# Autodesk Inventor assembly: DayLightGlow_DisplayPanel
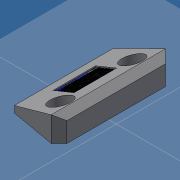
[picture p0: Inventor's stored thumbnail of the model, 180x180]
Saved by Autodesk Inventor 2019 (Build 230136000, 136)
## iProperties
Created: 2019-01-06
Part Number: DayLightGlow_DisplayPanel
Material: Generisch
Document SubType Name: Assembly
Designer: Stefan
Mass: 14.7018 g
Surface Area: 181.288 cm^2
Volume: 14.7018 cm^3
Density: 1 g/cm^3
Author: Stefan
## Documents named in this file (3)
- C:\Users\User\Documents\Inventor\DayLightGlow\DayLightGlow_DisplayPanel.iam
- C:\Users\User\Documents\Inventor\DayLightGlow\DayLightGlow_DisplayPanel.ipt
- C:\Users\User\Documents\Inventor\DayLightGlow\Geekcreit 1.3 Inch 4Pin.ipt
## Components (2 placed, 2 different names)
1. DayLightGlow_DisplayPanel:1 — Passend:1, Passend:2, Passend:3
2. Geekcreit 1.3 Inch 4Pin:1 — Passend:1, Passend:2, Passend:3
## Relationships (3: Mate 3)
- Passend:1 [Mate]: DayLightGlow_DisplayPanel:1 ↔ Geekcreit 1.3 Inch 4Pin:1
- Passend:2 [Mate]: DayLightGlow_DisplayPanel:1 ↔ Geekcreit 1.3 Inch 4Pin:1
- Passend:3 [Mate]: DayLightGlow_DisplayPanel:1 ↔ Geekcreit 1.3 Inch 4Pin:1
